# Autodesk Inventor assembly: Bucket_Final_Offset
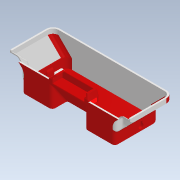
[picture p0: Inventor's stored thumbnail of the model, 180x180]
Saved by Autodesk Inventor 2022.1 (Build 261234020, 234B)
## iProperties
Created: 2022-07-24
Part Number: Bucket_Final_Offset
Document SubType Name: Assembly
Designer: Rama
Author: Rama
## Documents named in this file (3)
- C:\Users\Rama\Desktop\GitHub\Voron-2-Mods\Mandalaroseworks\BedPan\CAD\SRC\Bucket\Bucket_Offset.iam
- C:\Users\Rama\Desktop\GitHub\Voron-2-Mods\Mandalaroseworks\BedPan\CAD\SRC\Bucket\Bucket_Offset1.ipt
- C:\Users\Rama\Desktop\GitHub\Voron-2-Mods\Mandalaroseworks\BedPan\CAD\SRC\Bucket\Bucket_Offset2.ipt
## Components (2 placed, 2 different names)
1. Bucket_Offset1:1 — Fluchtend:1, Fluchtend:2, Passend:1
2. Bucket_Offset2:1 — Fluchtend:1, Fluchtend:2, Passend:1
## Relationships (3: Flush 2, Mate 1)
- Fluchtend:1 [Flush]: Bucket_Offset1:1 ↔ Bucket_Offset2:1
- Fluchtend:2 [Flush]: Bucket_Offset1:1 ↔ Bucket_Offset2:1
- Passend:1 [Mate] (-1 mm): Bucket_Offset1:1 ↔ Bucket_Offset2:1
